# Autodesk Inventor assembly: MotorHenkan
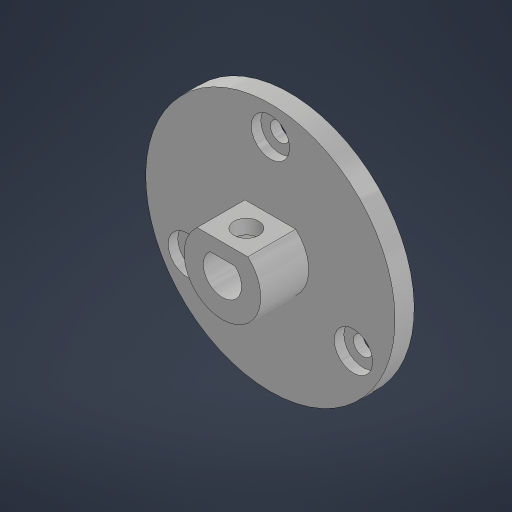
[picture p0: Inventor's stored thumbnail of the model, 512x512]
Saved by Autodesk Inventor 2024.2 (Build 282272000, 272)
## iProperties
Created: 2024-03-02
Part Number: MotorHenkan
Document SubType Name: Assembly
Designer: Hanaoka
Author: Hanaoka
## Documents named in this file (2)
- G:\共有ドライブ\reRo\05_個人\hanaoka\inventor\CAMpath\MotorHenkan.iam
- G:\共有ドライブ\reRo\05_個人\hanaoka\inventor\DriveUnit\Henkan\Henkan.ipt
## Components (1 placed, 1 different names)
1. Henkan:1 — メイト:1, 正接:1
## Relationships (2: Mate 1, Tangent 1)
- メイト:1 [Mate]: Henkan:1
- 正接:1 [Tangent]: Henkan:1
